# Autodesk Inventor assembly: złożenie nr1
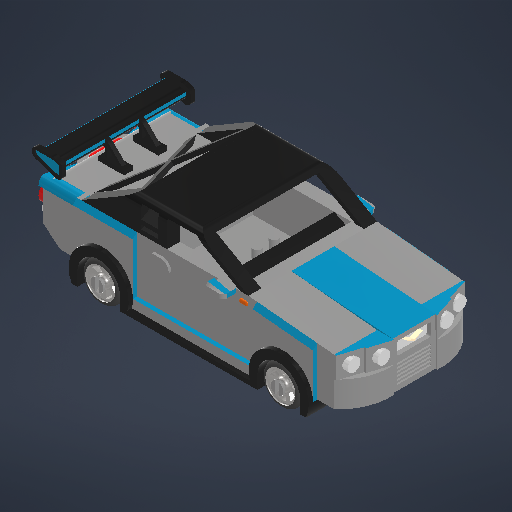
[picture p0: Inventor's stored thumbnail of the model, 512x512]
Saved by Autodesk Inventor 2026.2 (Build 302298000, 298)
## iProperties
Created: 2026-08-16
Part Number: złożenie nr1
Document SubType Name: Assembly
Designer: wojsl
Author: wojsl
## Documents named in this file (6)
- C:\Users\wojsl\OneDrive\Pulpit\cad\samochód\złożenie nr1.iam
- C:\Users\wojsl\OneDrive\Pulpit\cad\samochód\main.ipt
- C:\Users\wojsl\OneDrive\Pulpit\cad\samochód\opona.ipt
- C:\Users\wojsl\OneDrive\Pulpit\cad\samochód\zderzak.ipt
- C:\Users\wojsl\OneDrive\Pulpit\cad\samochód\dach.ipt
- C:\Users\wojsl\OneDrive\Pulpit\cad\samochód\spoiler.ipt
## Components (8 placed, 5 different names)
1. main:1 — Wstawiające:1, Wstawiające:2, Wstawiające:3, Wstawiające:4, Wstawiające:5, Wstawiające:6, Wstawiające:7, Wstawiające:8
2. opona:1 — Wstawiające:4
3. opona:2 — Wstawiające:3
4. opona:3 — Wstawiające:2
5. opona:4 — Wstawiające:1
6. zderzak:1 — Wstawiające:5, Wstawiające:6, Wstawiające:9, Wstawiające:10
7. dach:1 — Wstawiające:7, Wstawiające:8
8. spoiler:1 — Wstawiające:9, Wstawiające:10
## Relationships (10: Insert 10)
- Wstawiające:1 [Insert]: main:1 ↔ opona:4
- Wstawiające:2 [Insert]: main:1 ↔ opona:3
- Wstawiające:3 [Insert]: main:1 ↔ opona:2
- Wstawiające:4 [Insert]: main:1 ↔ opona:1
- Wstawiające:5 [Insert]: main:1 ↔ zderzak:1
- Wstawiające:6 [Insert]: main:1 ↔ zderzak:1
- Wstawiające:7 [Insert]: main:1 ↔ dach:1
- Wstawiające:8 [Insert]: main:1 ↔ dach:1
- Wstawiające:9 [Insert]: zderzak:1 ↔ spoiler:1
- Wstawiające:10 [Insert]: zderzak:1 ↔ spoiler:1
